# Autodesk Inventor assembly: dis
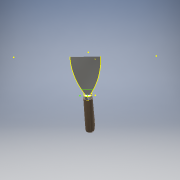
[picture p0: Inventor's stored thumbnail of the model, 180x180]
Saved by Autodesk Inventor 2018 (Build 220112000, 112)
## iProperties
Created: 2019-04-30
Part Number: dis
Document SubType Name: Assembly
Designer: russd
Author: russd
## Documents named in this file (4)
- C:\Users\10043883\Documents\GitHub\IED-files\dis.iam
- C:\Users\10043883\Documents\GitHub\IED-files\Dis.ipt
- C:\Users\10043883\Documents\GitHub\IED-files\dis1.ipt
- C:\Users\10043883\Documents\GitHub\IED-files\dis3.ipt
## Components (3 placed, 3 different names)
1. dis1:1 — Mate:1, Cylindrical:1, Mate:2
2. dis3:1 — Mate:1, Cylindrical:1
3. Dis:1 — Mate:2
## Relationships (3: Mate 2, CylindricalJoint 1)
- Mate:1: dis1:1 ↔ dis3:1
- Cylindrical:1: dis1:1 ↔ dis3:1
- Mate:2: dis1:1 ↔ Dis:1
